# Autodesk Inventor assembly: force_sensor_pcb_assy
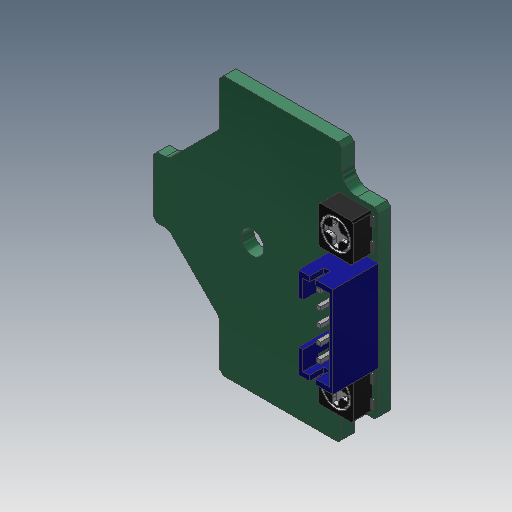
[picture p0: Inventor's stored thumbnail of the model, 512x512]
Saved by Autodesk Inventor 2019.4 (Build 234330000, 330)
## iProperties
Created: 2018-10-05
Part Number: force_sensor_pcb_assy
Material: 一般
Document SubType Name: Assembly
Designer: student
Author: student
## Documents named in this file (4)
- C:\Workspace\Yunit8-HaptHexa\Hardware\Inventor\Tibia\force_sensor_pcb_assy.iam
- C:\Workspace\Yunit8-HaptHexa\Hardware\Inventor\Tibia\force_sensor_pcb.ipt
- C:\Workspace\Yunit8-HaptHexa\Hardware\Inventor\Tibia\B5B-PH-K-S.ipt
- C:\Workspace\Yunit8-HaptHexa\Hardware\Inventor\Tibia\TOCOS G43A.ipt
## Components (4 placed, 3 different names)
1. force_sensor_pcb:1 — メイト:1, フラッシュ:1, メイト:2, フラッシュ:2, メイト:3, フラッシュ:3
2. B5B-PH-K-S:1 — メイト:1, フラッシュ:1
3. TOCOS G43A:1 — メイト:2, フラッシュ:2
4. TOCOS G43A:2 — メイト:3, フラッシュ:3
## Relationships (6: Mate 3, Flush 3)
- メイト:1 [Mate]: force_sensor_pcb:1 ↔ B5B-PH-K-S:1
- フラッシュ:1 [Flush]: force_sensor_pcb:1 ↔ B5B-PH-K-S:1
- メイト:2 [Mate]: force_sensor_pcb:1 ↔ TOCOS G43A:1
- フラッシュ:2 [Flush] (0.5 mm): force_sensor_pcb:1 ↔ TOCOS G43A:1
- メイト:3 [Mate]: force_sensor_pcb:1 ↔ TOCOS G43A:2
- フラッシュ:3 [Flush] (0.5 mm): force_sensor_pcb:1 ↔ TOCOS G43A:2
